# Autodesk Inventor assembly: SoporteBobina_2
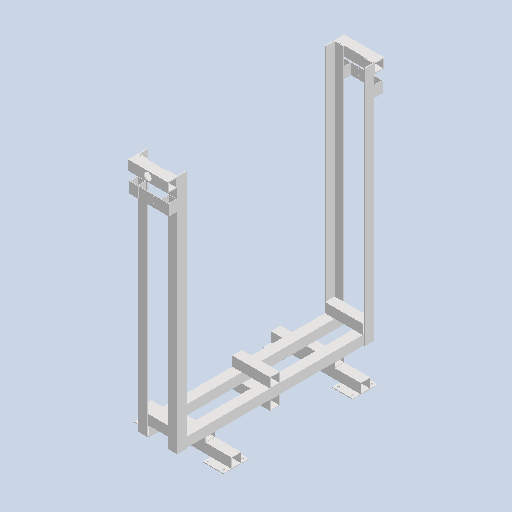
[picture p0: Inventor's stored thumbnail of the model, 512x512]
Saved by Autodesk Inventor 2022 (Build 260153000, 153)
## iProperties
Created: 2022-03-28
Part Number: SoporteBobina_2
Document SubType Name: Assembly
Designer: aarco
Author: aarco
## Documents named in this file (10)
- C:\Users\dovalle\OneDrive - ALTER TECHNOLOGY TÜV NORD, S.A.U\Escritorio\IDOM\REV_3\SoporteBobina_2.iam
- C:\Users\dovalle\OneDrive - ALTER TECHNOLOGY TÜV NORD, S.A.U\Escritorio\IDOM\REV_3\C_370_40_2.ipt
- C:\Users\dovalle\OneDrive - ALTER TECHNOLOGY TÜV NORD, S.A.U\Escritorio\IDOM\REV_3\C_156_40_2.ipt
- C:\Users\dovalle\OneDrive - ALTER TECHNOLOGY TÜV NORD, S.A.U\Escritorio\IDOM\REV_3\C_805_40_2.ipt
- C:\Users\dovalle\OneDrive - ALTER TECHNOLOGY TÜV NORD, S.A.U\Escritorio\IDOM\REV_3\Placa_Rueda_105x85_80x60_3.ipt
- C:\Users\dovalle\OneDrive - ALTER TECHNOLOGY TÜV NORD, S.A.U\Escritorio\IDOM\REV_3\A_992_40_4.ipt
- C:\Users\dovalle\OneDrive - ALTER TECHNOLOGY TÜV NORD, S.A.U\Escritorio\IDOM\REV_3\C_156_40_20_2.ipt
- C:\Users\dovalle\OneDrive - ALTER TECHNOLOGY TÜV NORD, S.A.U\Escritorio\IDOM\REV_3\C_164_40_4.ipt
- C:\Users\dovalle\OneDrive - ALTER TECHNOLOGY TÜV NORD, S.A.U\Escritorio\IDOM\REV_3\C_45_35_2.ipt
- C:\Users\dovalle\OneDrive - ALTER TECHNOLOGY TÜV NORD, S.A.U\Escritorio\IDOM\REV_3\PlacaSTC-HH20.ipt
## Components (26 placed, 9 different names)
1. C_370_40_2:1 — Rígido:16, Rígido:19, Rígido:27
2. C_370_40_2:2 — Rígido:17, Rígido:18, Rígido:26
3. C_156_40_2:1 — Rígido:1, Rígido:2
4. C_156_40_2:4 — Rígido:5
5. C_156_40_2:5 — Rígido:6
6. C_156_40_2:6 — Rígido:7
7. C_805_40_2:1 — Rígido:2, Rígido:6, Rígido:7, Rígido:22, Rígido:23, Coincidencia:1
8. C_805_40_2:2 — Rígido:1, Rígido:5, Rígido:20, Rígido:21, Nivelación:1, Coincidencia:2, Nivelación:4
9. Placa_Rueda_105x85_80x60_3:1 — Rígido:16
10. Placa_Rueda_105x85_80x60_3:2 — Rígido:17
11. Placa_Rueda_105x85_80x60_3:3 — Rígido:18
12. Placa_Rueda_105x85_80x60_3:4 — Rígido:19
13. A_992_40_4:1 — Rígido:20, Nivelación:3, Rígido:29, Coincidencia:7, Nivelación:9
14. A_992_40_4:2 — Rígido:22, Rígido:28, Coincidencia:4, Nivelación:8
15. A_992_40_4:3 — Rígido:23, Coincidencia:6, Nivelación:10
16. A_992_40_4:4 — Rígido:21, Nivelación:2, Coincidencia:3, Nivelación:5
17. C_156_40_20_2:1 — Rígido:26, Coincidencia:1, Nivelación:1, Nivelación:2
18. C_156_40_20_2:2 — Rígido:27, Coincidencia:2, Nivelación:3, Nivelación:4
19. C_164_40_4:1 — Rígido:29
20. C_164_40_4:2 — Rígido:28, Coincidencia:5
21. C_45_35_2:1 — Coincidencia:4, Nivelación:7, Coincidencia:5, Nivelación:8, Nivelación:12, Rígido:30
22. C_45_35_2:2 — Coincidencia:3, Nivelación:5, Nivelación:7
23. C_45_35_2:3 — Coincidencia:6, Nivelación:10, Nivelación:11, Nivelación:12
24. C_45_35_2:4 — Coincidencia:7, Nivelación:9, Nivelación:11, Rígido:31
25. PlacaSTC-HH20:1 — Rígido:31
26. PlacaSTC-HH20:2 — Rígido:30
## Relationships (37: WeldJoint 19, Flush 11, Mate 7)
- Rígido:1 [WeldJoint]: C_156_40_2:1 ↔ C_805_40_2:2
- Rígido:2 [WeldJoint]: C_156_40_2:1 ↔ C_805_40_2:1
- Rígido:5 [WeldJoint]: C_156_40_2:4 ↔ C_805_40_2:2
- Rígido:6 [WeldJoint]: C_156_40_2:5 ↔ C_805_40_2:1
- Rígido:7 [WeldJoint]: C_156_40_2:6 ↔ C_805_40_2:1
- Rígido:16 [WeldJoint]: C_370_40_2:1 ↔ Placa_Rueda_105x85_80x60_3:1
- Rígido:17 [WeldJoint]: C_370_40_2:2 ↔ Placa_Rueda_105x85_80x60_3:2
- Rígido:18 [WeldJoint]: C_370_40_2:2 ↔ Placa_Rueda_105x85_80x60_3:3
- Rígido:19 [WeldJoint]: C_370_40_2:1 ↔ Placa_Rueda_105x85_80x60_3:4
- Rígido:20 [WeldJoint]: C_805_40_2:2 ↔ A_992_40_4:1
- Rígido:21 [WeldJoint]: C_805_40_2:2 ↔ A_992_40_4:4
- Rígido:22 [WeldJoint]: C_805_40_2:1 ↔ A_992_40_4:2
- Rígido:23 [WeldJoint]: C_805_40_2:1 ↔ A_992_40_4:3
- Rígido:26 [WeldJoint]: C_370_40_2:2 ↔ C_156_40_20_2:1
- Rígido:27 [WeldJoint]: C_370_40_2:1 ↔ C_156_40_20_2:2
- Coincidencia:1 [Mate]: C_805_40_2:1 ↔ C_156_40_20_2:1
- Nivelación:1 [Flush]: C_805_40_2:2 ↔ C_156_40_20_2:1
- Nivelación:2 [Flush] (120 mm): A_992_40_4:4 ↔ C_156_40_20_2:1
- Coincidencia:2 [Mate]: C_805_40_2:2 ↔ C_156_40_20_2:2
- Nivelación:3 [Flush] (120 mm): A_992_40_4:1 ↔ C_156_40_20_2:2
- Nivelación:4 [Flush]: C_805_40_2:2 ↔ C_156_40_20_2:2
- Rígido:28 [WeldJoint]: A_992_40_4:2 ↔ C_164_40_4:2
- Rígido:29 [WeldJoint]: A_992_40_4:1 ↔ C_164_40_4:1
- Coincidencia:3 [Mate]: A_992_40_4:4 ↔ C_45_35_2:2
- Coincidencia:4 [Mate]: A_992_40_4:2 ↔ C_45_35_2:1
- Nivelación:5 [Flush]: A_992_40_4:4 ↔ C_45_35_2:2
- Nivelación:7 [Flush]: C_45_35_2:1 ↔ C_45_35_2:2
- Coincidencia:5 [Mate] (39.5 mm): C_164_40_4:2 ↔ C_45_35_2:1
- Coincidencia:6 [Mate]: A_992_40_4:3 ↔ C_45_35_2:3
- Coincidencia:7 [Mate]: A_992_40_4:1 ↔ C_45_35_2:4
- Nivelación:8 [Flush]: A_992_40_4:2 ↔ C_45_35_2:1
- Nivelación:9 [Flush]: A_992_40_4:1 ↔ C_45_35_2:4
- Nivelación:10 [Flush]: A_992_40_4:3 ↔ C_45_35_2:3
- Nivelación:11 [Flush]: C_45_35_2:3 ↔ C_45_35_2:4
- Nivelación:12 [Flush]: C_45_35_2:1 ↔ C_45_35_2:3
- Rígido:30 [WeldJoint]: C_45_35_2:1 ↔ PlacaSTC-HH20:2
- Rígido:31 [WeldJoint]: C_45_35_2:4 ↔ PlacaSTC-HH20:1
